# Autodesk Inventor assembly: EnsamblajeMoto
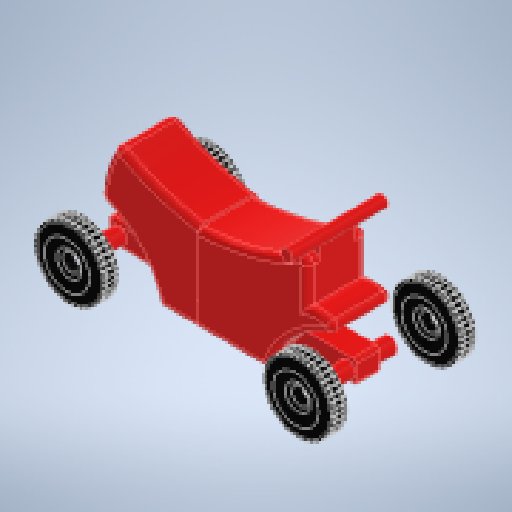
[picture p0: Inventor's stored thumbnail of the model, 512x512]
Saved by Autodesk Inventor 2025.1 (Build 291241000, 241)
## iProperties
Created: 2025-01-19
Part Number: EnsamblajeMoto
Document SubType Name: Assembly
Designer: usuario
Author: usuario
## Documents named in this file (4)
- C:\Users\yovan\Desktop\APM\ausol-apm.github.io\project\Design and simulation\Inventor\Modelado juguetes\Cad Juguetes\Moto\EnsamblajeMoto.iam
- C:\Users\yovan\Desktop\APM\ausol-apm.github.io\project\Design and simulation\Inventor\Modelado juguetes\Cad Juguetes\Moto\PiezaParteAtrasMoto.ipt
- C:\Users\yovan\Desktop\APM\ausol-apm.github.io\project\Design and simulation\Inventor\Modelado juguetes\Cad Juguetes\Moto\Llanta.ipt
- C:\Users\yovan\Desktop\APM\ausol-apm.github.io\project\Design and simulation\Inventor\Modelado juguetes\Cad Juguetes\Moto\PiezaParteDelanteraMoto.ipt
## Components (6 placed, 3 different names)
1. PiezaParteAtrasMoto:1 — Mate:1, Flush:1, Flush:2, Insert:1, Insert:4
2. Llanta:1 — Insert:1
3. Llanta:2 — Insert:2
4. Llanta:3 — Insert:3
5. Llanta:4 — Insert:4
6. PiezaParteDelanteraMoto:1 — Mate:1, Flush:1, Flush:2, Insert:2, Insert:3
## Relationships (7: Insert 4, Flush 2, Mate 1)
- Mate:1: PiezaParteAtrasMoto:1 ↔ PiezaParteDelanteraMoto:1
- Flush:1: PiezaParteAtrasMoto:1 ↔ PiezaParteDelanteraMoto:1
- Flush:2: PiezaParteAtrasMoto:1 ↔ PiezaParteDelanteraMoto:1
- Insert:1 (10 mm): PiezaParteAtrasMoto:1 ↔ Llanta:1
- Insert:2 (10 mm): Llanta:2 ↔ PiezaParteDelanteraMoto:1
- Insert:3 (20 mm): Llanta:3 ↔ PiezaParteDelanteraMoto:1
- Insert:4 (20 mm): PiezaParteAtrasMoto:1 ↔ Llanta:4
